# Autodesk Inventor assembly: FullField-ver3-1111-2021
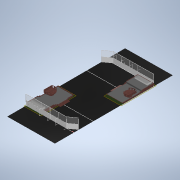
[picture p0: Inventor's stored thumbnail of the model, 180x180]
Saved by Autodesk Inventor 2021 (Build 250183000, 183)
## iProperties
Created: 2021-02-23
Part Number: FullField-ver3-1111-2021
Document SubType Name: Assembly
Designer: CMurray
Author: CMurray
## Documents named in this file (9)
- F:\PHRC CADD 2021\2021 Game Design Challenge\Full Field\Final Assembly\FullField-ver3-1111-2021.iam
- F:\PHRC CADD 2021\2021 Game Design Challenge\Full Field\Parts\FieldFloor-ver1-1111-2021.ipt
- F:\PHRC CADD 2021\2021 Game Design Challenge\Full Field\Parts\Tape\Tape.ipt
- F:\PHRC CADD 2021\2021 Game Design Challenge\Full Field\Parts\Tape\RedAllianceTape-ver1-1111-2021.ipt
- F:\PHRC CADD 2021\2021 Game Design Challenge\Full Field\Parts\Tape\BlueAllianceTape-ver1-1111-2021.ipt
- F:\PHRC CADD 2021\2021 Game Design Challenge\Main Ship\ShipDesign-ver4-1111-2021.ipt
- F:\PHRC CADD 2021\2021 Game Design Challenge\Misc\ShootingBox-ver1-1111-2021.ipt
- F:\PHRC CADD 2021\2021 Game Design Challenge\Player Station\Assemblies\DriverStation-ver2-1111-2021.iam
- F:\PHRC CADD 2021\2021 Game Design Challenge\Crow's Nest\Assemblies\CrowsNestFinal-ver3-1111-2021.iam
## Components (18 placed, 8 different names)
1. FieldFloor-ver1-1111-2021:1 — Flush:1, Flush:2, Mate:1, Mate:3, Mate:10, Flush:10, Mate:14, Flush:12, Mate:16, Flush:15, Mate:32, Mate:34
2. FieldFloor-ver1-1111-2021:2 — Flush:1, Flush:2, Mate:1, Mate:2, Flush:3, Flush:4, Flush:5, Flush:6, Mate:4, Flush:7, Mate:6, Flush:8, Mate:8, Flush:9, Mate:12, Flush:11, Mate:17, Flush:16, Flush:19
3. ShipDesign-ver4-1111-2021:1 — Mate:16, Mate:24, Mate:25, Mate:26, Flush:15, Flush:18, Mate:36, Mate:38, Flush:20
4. ShipDesign-ver4-1111-2021:2 — Mate:17, Flush:16, Mate:29, Mate:30, Mate:31, Mate:37, Mate:39, Flush:21
5. ShootingBox-ver1-1111-2021:1 — Mate:24, Mate:25, Mate:26
6. ShootingBox-ver1-1111-2021:2 — Mate:29, Mate:30, Mate:31
7. DriverStation-ver2-1111-2021:1 [sub-assembly] — Mate:32, Flush:18, Mate:33, Mate:36
8. DriverStation-ver2-1111-2021:2 [sub-assembly] — Mate:34, Mate:35, Flush:19, Mate:37
9. CrowsNestFinal-ver3-1111-2021:1 [sub-assembly] — Mate:38, Flush:20
10. CrowsNestFinal-ver3-1111-2021:2 [sub-assembly] — Mate:39, Flush:21
11. Tape:1 — Mate:2, Flush:3, Flush:4, Mate:5, Mate:9, Mate:11, Mate:33
12. Tape:2 — Mate:3, Flush:5, Flush:6, Mate:7, Mate:13, Mate:15, Mate:35
13. Tape:3 — Mate:4, Flush:7, Mate:5
14. Tape:4 — Mate:6, Flush:8, Mate:7
15. RedAllianceTape-ver1-1111-2021:1 — Mate:8, Flush:9, Mate:9
16. RedAllianceTape-ver1-1111-2021:2 — Mate:10, Flush:10, Mate:11
17. BlueAllianceTape-ver1-1111-2021:1 — Mate:12, Flush:11, Mate:13
18. BlueAllianceTape-ver1-1111-2021:2 — Mate:14, Flush:12, Mate:15
## Relationships (49: Mate 31, Flush 18)
- Flush:1: FieldFloor-ver1-1111-2021:1 ↔ FieldFloor-ver1-1111-2021:2
- Flush:2: FieldFloor-ver1-1111-2021:1 ↔ FieldFloor-ver1-1111-2021:2
- Mate:1: FieldFloor-ver1-1111-2021:1 ↔ FieldFloor-ver1-1111-2021:2
- Mate:2: FieldFloor-ver1-1111-2021:2 ↔ Tape:1
- Flush:3: FieldFloor-ver1-1111-2021:2 ↔ Tape:1
- Flush:4 (3606.8 mm): FieldFloor-ver1-1111-2021:2 ↔ Tape:1
- Mate:3: FieldFloor-ver1-1111-2021:1 ↔ Tape:2
- Flush:5: FieldFloor-ver1-1111-2021:2 ↔ Tape:2
- Flush:6 (3606.8 mm): FieldFloor-ver1-1111-2021:2 ↔ Tape:2
- Mate:4: FieldFloor-ver1-1111-2021:2 ↔ Tape:3
- Flush:7: FieldFloor-ver1-1111-2021:2 ↔ Tape:3
- Mate:5 (3657.6 mm): Tape:1 ↔ Tape:3
- Mate:6: FieldFloor-ver1-1111-2021:2 ↔ Tape:4
- Flush:8: FieldFloor-ver1-1111-2021:2 ↔ Tape:4
- Mate:7 (3657.6 mm): Tape:2 ↔ Tape:4
- Mate:8: FieldFloor-ver1-1111-2021:2 ↔ RedAllianceTape-ver1-1111-2021:1
- Flush:9: FieldFloor-ver1-1111-2021:2 ↔ RedAllianceTape-ver1-1111-2021:1
- Mate:9: Tape:1 ↔ RedAllianceTape-ver1-1111-2021:1
- Mate:10: FieldFloor-ver1-1111-2021:1 ↔ RedAllianceTape-ver1-1111-2021:2
- Flush:10: FieldFloor-ver1-1111-2021:1 ↔ RedAllianceTape-ver1-1111-2021:2
- Mate:11: Tape:1 ↔ RedAllianceTape-ver1-1111-2021:2
- Mate:12: FieldFloor-ver1-1111-2021:2 ↔ BlueAllianceTape-ver1-1111-2021:1
- Flush:11: FieldFloor-ver1-1111-2021:2 ↔ BlueAllianceTape-ver1-1111-2021:1
- Mate:13: Tape:2 ↔ BlueAllianceTape-ver1-1111-2021:1
- Mate:14: FieldFloor-ver1-1111-2021:1 ↔ BlueAllianceTape-ver1-1111-2021:2
- Flush:12: FieldFloor-ver1-1111-2021:1 ↔ BlueAllianceTape-ver1-1111-2021:2
- Mate:15: Tape:2 ↔ BlueAllianceTape-ver1-1111-2021:2
- Mate:16: FieldFloor-ver1-1111-2021:1 ↔ ShipDesign-ver4-1111-2021:1
- Mate:17: FieldFloor-ver1-1111-2021:2 ↔ ShipDesign-ver4-1111-2021:2
- Mate:24: ShipDesign-ver4-1111-2021:1 ↔ ShootingBox-ver1-1111-2021:1
- Mate:25: ShipDesign-ver4-1111-2021:1 ↔ ShootingBox-ver1-1111-2021:1
- Mate:26 (254 mm): ShipDesign-ver4-1111-2021:1 ↔ ShootingBox-ver1-1111-2021:1
- Flush:15: FieldFloor-ver1-1111-2021:1 ↔ ShipDesign-ver4-1111-2021:1
- Flush:16: FieldFloor-ver1-1111-2021:2 ↔ ShipDesign-ver4-1111-2021:2
- Mate:29: ShipDesign-ver4-1111-2021:2 ↔ ShootingBox-ver1-1111-2021:2
- Mate:30: ShipDesign-ver4-1111-2021:2 ↔ ShootingBox-ver1-1111-2021:2
- Mate:31 (254 mm): ShipDesign-ver4-1111-2021:2 ↔ ShootingBox-ver1-1111-2021:2
- Mate:32: FieldFloor-ver1-1111-2021:1 ↔ DriverStation-ver2-1111-2021:1
- Flush:18 (3048 mm): ShipDesign-ver4-1111-2021:1 ↔ DriverStation-ver2-1111-2021:1
- Mate:33: DriverStation-ver2-1111-2021:1 ↔ Tape:1
- Mate:34: FieldFloor-ver1-1111-2021:1 ↔ DriverStation-ver2-1111-2021:2
- Mate:35: DriverStation-ver2-1111-2021:2 ↔ Tape:2
- Flush:19: FieldFloor-ver1-1111-2021:2 ↔ DriverStation-ver2-1111-2021:2
- Mate:36: ShipDesign-ver4-1111-2021:1 ↔ DriverStation-ver2-1111-2021:1
- Mate:37: ShipDesign-ver4-1111-2021:2 ↔ DriverStation-ver2-1111-2021:2
- Mate:38: ShipDesign-ver4-1111-2021:1 ↔ CrowsNestFinal-ver3-1111-2021:1
- Flush:20: ShipDesign-ver4-1111-2021:1 ↔ CrowsNestFinal-ver3-1111-2021:1
- Mate:39: ShipDesign-ver4-1111-2021:2 ↔ CrowsNestFinal-ver3-1111-2021:2
- Flush:21: ShipDesign-ver4-1111-2021:2 ↔ CrowsNestFinal-ver3-1111-2021:2
